# Autodesk Inventor assembly: prostkatna szeroka wysoka kwadraty
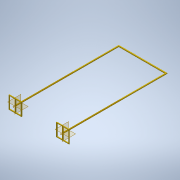
[picture p0: Inventor's stored thumbnail of the model, 180x180]
Saved by Autodesk Inventor 2021 (Build 250183000, 183)
## iProperties
Created: 2024-04-18
Part Number: prostkatna szeroka wysoka kwadraty
Document SubType Name: Assembly
Designer: Michal
Author: Michal
## Documents named in this file (8)
- C:\Users\Michal\Documents\GitHub\PNW_PhotoBoothFrame_3D\prostkatna szeroka wysoka kwadraty.iam
- C:\Users\Michal\Documents\GitHub\PNW_PhotoBoothFrame_3D\Gora L1500.ipt
- C:\Users\Michal\Documents\GitHub\PNW_PhotoBoothFrame_3D\Naroznik.iam
- C:\Users\Michal\Documents\GitHub\PNW_PhotoBoothFrame_3D\Stopa v1.iam
- C:\Users\Michal\Documents\GitHub\PNW_PhotoBoothFrame_3D\Noga L L1600.ipt
- C:\Users\Michal\Documents\GitHub\PNW_PhotoBoothFrame_3D\Noga P L1600.ipt
- C:\Users\Michal\Documents\GitHub\PNW_PhotoBoothFrame_3D\Lacznik prosty sruby.iam
- C:\Users\Michal\Documents\GitHub\PNW_PhotoBoothFrame_3D\Przedluzka L1500.ipt
## Components (11 placed, 7 different names)
1. Stopa v1:1 [sub-assembly] — Flush:1, Flush:2, Flush:3, Mate:2, Mate:40, Flush:8, Flush:9
2. Stopa v1:2 [sub-assembly] — Flush:1, Flush:2, Flush:4, Flush:5, Mate:11, Mate:41, Flush:10, Flush:11
3. Naroznik:1 [sub-assembly] — Mate:12, Mate:13, Mate:14, Mate:15
4. Naroznik:2 [sub-assembly] — Mate:7, Mate:8, Mate:9, Mate:17
5. Noga L L1600:1 — Flush:3, Mate:2, Mate:7, Mate:8, Mate:9, Mate:47
6. Noga P L1600:1 — Flush:4, Flush:5, Mate:11, Mate:12, Mate:13, Mate:14, Flush:6, Mate:48
7. Gora L1500:1 — Flush:6, Mate:15, Mate:17, Mate:38, Flush:7, Mate:39
8. Lacznik prosty sruby:1 [sub-assembly] — Flush:12, Mate:42, Mate:43, Mate:47
9. Przedluzka L1500:1 — Mate:40, Flush:8, Flush:9, Flush:12, Mate:42, Mate:43
10. Przedluzka L1500:2 — Mate:41, Flush:10, Flush:11, Mate:44, Mate:45, Mate:46
11. Lacznik prosty sruby:2 [sub-assembly] — Mate:44, Mate:45, Mate:46, Mate:48
## Relationships (33: Mate 21, Flush 12)
- Flush:1: Stopa v1:1 ↔ Stopa v1:2
- Flush:2: Stopa v1:1 ↔ Stopa v1:2
- Flush:3: Stopa v1:1 ↔ Noga L L1600:1
- Mate:2: Stopa v1:1 ↔ Noga L L1600:1
- Mate:7: Naroznik:2 ↔ Noga L L1600:1
- Mate:8: Naroznik:2 ↔ Noga L L1600:1
- Mate:9: Naroznik:2 ↔ Noga L L1600:1
- Flush:4: Stopa v1:2 ↔ Noga P L1600:1
- Flush:5: Stopa v1:2 ↔ Noga P L1600:1
- Mate:11: Stopa v1:2 ↔ Noga P L1600:1
- Mate:12: Naroznik:1 ↔ Noga P L1600:1
- Mate:13: Naroznik:1 ↔ Noga P L1600:1
- Mate:14: Naroznik:1 ↔ Noga P L1600:1
- Flush:6: Noga P L1600:1 ↔ Gora L1500:1
- Mate:15: Naroznik:1 ↔ Gora L1500:1
- Mate:17: Naroznik:2 ↔ Gora L1500:1
- Mate:38: Gora L1500:1
- Flush:7: Gora L1500:1
- Mate:39: Gora L1500:1
- Mate:40: Stopa v1:1 ↔ Przedluzka L1500:1
- Flush:8: Stopa v1:1 ↔ Przedluzka L1500:1
- Flush:9: Stopa v1:1 ↔ Przedluzka L1500:1
- Mate:41: Stopa v1:2 ↔ Przedluzka L1500:2
- Flush:10: Stopa v1:2 ↔ Przedluzka L1500:2
- Flush:11: Stopa v1:2 ↔ Przedluzka L1500:2
- Flush:12: Lacznik prosty sruby:1 ↔ Przedluzka L1500:1
- Mate:42: Lacznik prosty sruby:1 ↔ Przedluzka L1500:1
- Mate:43: Lacznik prosty sruby:1 ↔ Przedluzka L1500:1
- Mate:44: Przedluzka L1500:2 ↔ Lacznik prosty sruby:2
- Mate:45: Przedluzka L1500:2 ↔ Lacznik prosty sruby:2
- Mate:46: Przedluzka L1500:2 ↔ Lacznik prosty sruby:2
- Mate:47: Noga L L1600:1 ↔ Lacznik prosty sruby:1
- Mate:48: Noga P L1600:1 ↔ Lacznik prosty sruby:2
